# Autodesk Inventor assembly: Assembly of Bot
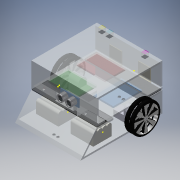
[picture p0: Inventor's stored thumbnail of the model, 180x180]
Saved by Autodesk Inventor 2018 (Build 220112000, 112)
## iProperties
Created: 2018-02-19
Part Number: Assembly of Bot
Document SubType Name: Assembly
Designer: Melda
Author: Melda
## Documents named in this file (10)
- C:\Users\Melda\Desktop\SumoBot\Assembly of Bot.iam
- C:\Users\Melda\Desktop\SumoBot\Bottom Plastic.ipt
- C:\Users\Melda\Desktop\SumoBot\Battery Box.ipt
- C:\Users\Melda\Desktop\SumoBot\Motor.ipt
- C:\Users\Melda\Desktop\SumoBot\Wheel.ipt
- C:\Users\Melda\Desktop\SumoBot\Velcro for Back.ipt
- C:\Users\Melda\Desktop\SumoBot\Stage with Boards.ipt
- C:\Users\Melda\Desktop\SumoBot\Flat Hinge.ipt
- C:\Users\Melda\Desktop\SumoBot\Top Plastic.ipt
- C:\Users\Melda\Desktop\SumoBot\Sonar.ipt
## Components (15 placed, 9 different names)
1. Bottom Plastic:1 — Flush:3, Mate:2, Flush:4, Mate:3, Mate:4, Flush:5, Flush:6, Flush:7, Flush:12, Flush:13, Mate:8, Mate:9, Flush:14, Flush:15, Mate:10, Mate:11, Flush:16, Flush:17, Flush:18, Flush:19, Mate:12, Flush:20, Flush:21, Mate:13, Flush:23, Mate:16, Flush:24
2. Battery Box:1 — Mate:2, Flush:23, Mate:16, Flush:25
3. Battery Box:2 — Flush:3, Flush:24, Flush:25
4. Motor:1 — Mate:4, Flush:5, Flush:6, Insert:3, Insert:4, Mate:13
5. Motor:2 — Flush:4, Mate:3, Flush:7, Insert:1, Insert:2
6. Wheel:1 — Insert:1
7. Wheel:2 — Insert:2
8. Wheel:3 — Insert:3
9. Wheel:4 — Insert:4
10. Velcro for Back:1 — Flush:12, Flush:13, Mate:9
11. Stage with Boards:1 — Mate:8, Flush:14, Flush:15
12. Flat Hinge:1 — Mate:10, Flush:17, Flush:18
13. Flat Hinge:2 — Mate:11, Flush:16, Flush:19
14. Top Plastic:1 — Mate:12, Flush:20, Flush:21, Mate:14, Mate:15, Flush:22
15. Sonar:1 — Mate:14, Mate:15, Flush:22
## Relationships (35: Flush 19, Mate 12, Insert 4)
- Flush:3 (4 mm): Bottom Plastic:1 ↔ Battery Box:2
- Mate:2: Bottom Plastic:1 ↔ Battery Box:1
- Flush:4: Bottom Plastic:1 ↔ Motor:2
- Mate:3: Bottom Plastic:1 ↔ Motor:2
- Mate:4: Bottom Plastic:1 ↔ Motor:1
- Flush:5: Bottom Plastic:1 ↔ Motor:1
- Flush:6 (50 mm): Bottom Plastic:1 ↔ Motor:1
- Flush:7 (50 mm): Bottom Plastic:1 ↔ Motor:2
- Insert:1 (8 mm): Motor:2 ↔ Wheel:1
- Insert:2: Motor:2 ↔ Wheel:2
- Insert:3 (8 mm): Motor:1 ↔ Wheel:3
- Insert:4: Motor:1 ↔ Wheel:4
- Flush:12 (1 mm): Bottom Plastic:1 ↔ Velcro for Back:1
- Flush:13: Bottom Plastic:1 ↔ Velcro for Back:1
- Mate:8: Bottom Plastic:1 ↔ Stage with Boards:1
- Mate:9: Bottom Plastic:1 ↔ Velcro for Back:1
- Flush:14 (19 mm): Bottom Plastic:1 ↔ Stage with Boards:1
- Flush:15: Bottom Plastic:1 ↔ Stage with Boards:1
- Mate:10: Bottom Plastic:1 ↔ Flat Hinge:1
- Mate:11: Bottom Plastic:1 ↔ Flat Hinge:2
- Flush:16 (30 mm): Bottom Plastic:1 ↔ Flat Hinge:2
- Flush:17 (30 mm): Bottom Plastic:1 ↔ Flat Hinge:1
- Flush:18 (21 mm): Bottom Plastic:1 ↔ Flat Hinge:1
- Flush:19 (21 mm): Bottom Plastic:1 ↔ Flat Hinge:2
- Mate:12: Bottom Plastic:1 ↔ Top Plastic:1
- Flush:20 (-1 mm): Bottom Plastic:1 ↔ Top Plastic:1
- Flush:21: Bottom Plastic:1 ↔ Top Plastic:1
- Mate:13: Bottom Plastic:1 ↔ Motor:1
- Mate:14: Top Plastic:1 ↔ Sonar:1
- Mate:15: Top Plastic:1 ↔ Sonar:1
- Flush:22: Top Plastic:1 ↔ Sonar:1
- Flush:23 (10 mm): Bottom Plastic:1 ↔ Battery Box:1
- Mate:16 (110 mm): Bottom Plastic:1 ↔ Battery Box:1
- Flush:24 (10 mm): Bottom Plastic:1 ↔ Battery Box:2
- Flush:25: Battery Box:1 ↔ Battery Box:2
